# Autodesk Inventor assembly: Assy_fork_connection
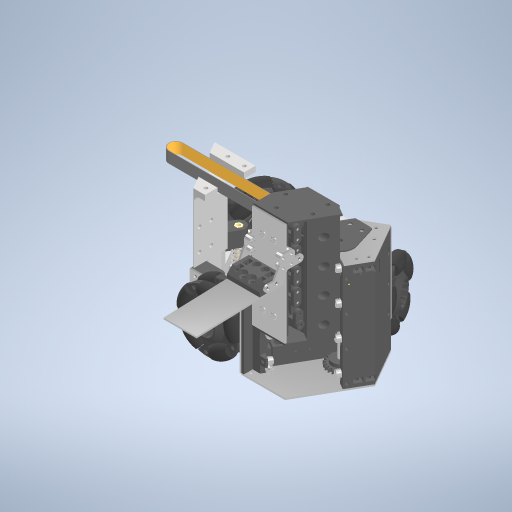
[picture p0: Inventor's stored thumbnail of the model, 512x512]
Saved by Autodesk Inventor 2024.1 (Build 281209000, 209)
## iProperties
Created: 2025-03-04
Part Number: Assy_fork_connection
Document SubType Name: Assembly
Designer: hibik
Author: hibik
## Documents named in this file (6)
- C:\Users\hibik\Documents\Robomech\RESCUE\ORCA\hard\Assy_fork_connection.iam
- C:\Users\hibik\Documents\Robomech\RESCUE\ORCA\hard\Assy_foot.iam
- C:\Users\hibik\Documents\Robomech\RESCUE\ORCA\hard\fork\right\Assy_fork_right.iam
- C:\Users\hibik\Documents\Robomech\RESCUE\ORCA\hard\flame_base\base2fork_connecter_front.ipt
- C:\Users\hibik\Documents\Robomech\RESCUE\ORCA\hard\flame_base\base2fork_connecter_back.ipt
- C:\Users\hibik\Documents\Robomech\RESCUE\ORCA\hard\fork\belt.ipt
## Components (5 placed, 5 different names)
1. Assy_foot:1 [sub-assembly] — 挿入:1, 挿入:2, 挿入:3, 挿入:4
2. Assy_fork_right:1 [sub-assembly] — 挿入:5, 挿入:6, 挿入:7
3. base2fork_connecter_back:1 — 挿入:1, 挿入:2, 挿入:6
4. base2fork_connecter_front:1 — 挿入:3, 挿入:4, 挿入:5
5. belt:1 — 挿入:7, 角度:1
## Relationships (8: Insert 7, Angle 1)
- 挿入:1 [Insert]: Assy_foot:1 ↔ base2fork_connecter_back:1
- 挿入:2 [Insert]: Assy_foot:1 ↔ base2fork_connecter_back:1
- 挿入:3 [Insert]: Assy_foot:1 ↔ base2fork_connecter_front:1
- 挿入:4 [Insert]: Assy_foot:1 ↔ base2fork_connecter_front:1
- 挿入:5 [Insert]: Assy_fork_right:1 ↔ base2fork_connecter_front:1
- 挿入:6 [Insert]: Assy_fork_right:1 ↔ base2fork_connecter_back:1
- 挿入:7 [Insert]: Assy_fork_right:1 ↔ belt:1
- 角度:1 [Angle] (0 deg): belt:1
